# Autodesk Inventor assembly: Assembly
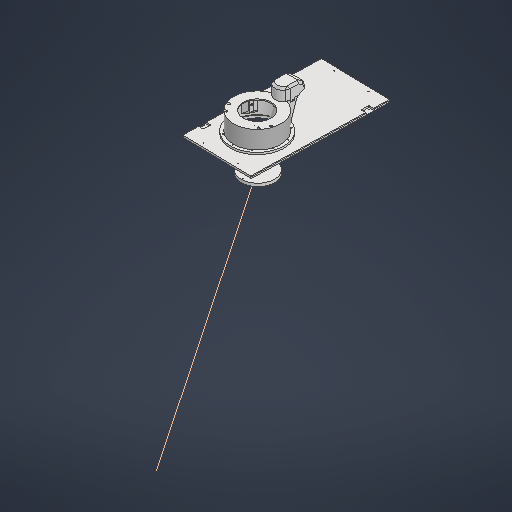
[picture p0: Inventor's stored thumbnail of the model, 512x512]
Saved by Autodesk Inventor 2026.1 (Build 301233000, 233)
## iProperties
Created: 2025-09-29
Part Number: Assembly
Document SubType Name: Assembly
Designer: mateo
Author: mateo
## Documents named in this file (6)
- C:\GitHub\In-situ-monitoring-of-powder-bed-fusion-additive-manufacturing\system_development\Mithril\v0.3\hardware_development\Assembly.iam
- C:\GitHub\In-situ-monitoring-of-powder-bed-fusion-additive-manufacturing\system_development\Mithril\v0.3\hardware_development\Cover Parts\flircamera+lens.ipt
- C:\GitHub\In-situ-monitoring-of-powder-bed-fusion-additive-manufacturing\system_development\Mithril\v0.3\hardware_development\Cover Parts\substrate plate.ipt
- C:\GitHub\In-situ-monitoring-of-powder-bed-fusion-additive-manufacturing\system_development\Mithril\v0.3\hardware_development\Cover Parts\12mm Cover.ipt
- C:\GitHub\In-situ-monitoring-of-powder-bed-fusion-additive-manufacturing\system_development\Mithril\v0.3\hardware_development\Cover Parts\lid - Copy.ipt
- C:\GitHub\In-situ-monitoring-of-powder-bed-fusion-additive-manufacturing\system_development\Mithril\v0.3\hardware_development\Cover Parts\Cylinder Housing Camera - Copy.ipt
## Components (5 placed, 5 different names)
1. flircamera+lens:1 — Mate:1, Mate:2, Mate:3
2. substrate plate:1 — Rotational:1
3. 12mm Cover:1 — Rotational:1, Insert:1
4. lid - Copy:1 — Mate:4, Mate:5, Mate:6
5. Cylinder Housing Camera - Copy:1 — Insert:1, Mate:2, Mate:3, Mate:4, Mate:5, Mate:6
## Relationships (8: Mate 6, RevoluteJoint 1, Insert 1)
- Mate:1: flircamera+lens:1
- Rotational:1 [RevoluteJoint] (-150 mm): substrate plate:1 ↔ 12mm Cover:1
- Insert:1: 12mm Cover:1 ↔ Cylinder Housing Camera - Copy:1
- Mate:2: flircamera+lens:1 ↔ Cylinder Housing Camera - Copy:1
- Mate:3: flircamera+lens:1 ↔ Cylinder Housing Camera - Copy:1
- Mate:4: lid - Copy:1 ↔ Cylinder Housing Camera - Copy:1
- Mate:5: lid - Copy:1 ↔ Cylinder Housing Camera - Copy:1
- Mate:6 (0.25 mm): lid - Copy:1 ↔ Cylinder Housing Camera - Copy:1
